# Autodesk Inventor assembly: Body
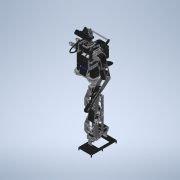
[picture p0: Inventor's stored thumbnail of the model, 180x180]
Saved by Autodesk Inventor 2020 (Build 240168000, 168)
## iProperties
Created: 2021-09-30
Part Number: Body
Document SubType Name: Assembly
Designer: Masato Kubotera
Mass: 4463.19 g
Surface Area: 13321.9 cm^2
Volume: 2213.37 cm^3
Density: 2.01647 g/cm^3
Author: Masato Kubotera
## Documents named in this file (3)
- C:\Users\Masato\Desktop\OpenPlatform_ver3_0 - Ver4_1branch\Body.iam
- C:\Users\Masato\Desktop\OpenPlatform_ver3_0 - Ver4_1branch\UpperBody\UpperBody.iam
- C:\Users\Masato\Desktop\OpenPlatform_ver3_0 - Ver4_1branch\LowerBody\LowerBody.iam
## Components (2 placed, 2 different names)
1. UpperBody:1 [sub-assembly] — 挿入:1
2. LowerBody:1 [sub-assembly] — 挿入:1, メイト:1
## Relationships (2: Insert 1, Mate 1)
- 挿入:1 [Insert]: UpperBody:1 ↔ LowerBody:1
- メイト:1 [Mate]: LowerBody:1
